# Autodesk Inventor assembly: LowerBody_MIR
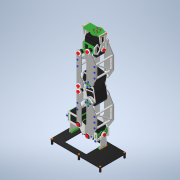
[picture p0: Inventor's stored thumbnail of the model, 180x180]
Saved by Autodesk Inventor 2020 (Build 240168000, 168)
## iProperties
Created: 2021-12-27
Part Number: LowerBody_MIR
Document SubType Name: Assembly
Designer: Masato Kubotera
Mass: 734.319 g
Surface Area: 2704.73 cm^2
Volume: 452.645 cm^3
Density: 1.62229 g/cm^3
Author: Masato Kubotera
## Documents named in this file (12)
- C:\Users\Masato\Desktop\OpenPlatform_ver3_0 - Ver4_1branch\LowerBody\LowerBody_MIR.iam
- C:\Users\Masato\Desktop\OpenPlatform_ver3_0 - Ver4_1branch\LowerBody\Leg_joit\Leg_joint_roll_yaw.iam
- C:\Users\Masato\Desktop\OpenPlatform_ver3_0 - Ver4_1branch\LowerBody\Leg_joit\Leg_joint_roll_pitch.iam
- C:\Users\Masato\Desktop\OpenPlatform_ver3_0 - Ver4_1branch\LowerBody\Slider_crank\Slider_crank_mechanism.iam
- C:\Users\Masato\Desktop\OpenPlatform_ver3_0 - Ver4_1branch\LowerBody\Link\FrontLink.iam
- C:\Users\Masato\Desktop\OpenPlatform_ver3_0 - Ver4_1branch\LowerBody\Link\BackUpperLink.iam
- C:\Users\Masato\Desktop\OpenPlatform_ver3_0 - Ver4_1branch\LowerBody\Link\BackLowerLink.iam
- C:\Users\Masato\Desktop\OpenPlatform_ver3_0 - Ver4_1branch\LowerBody\Ankle\Ankle_side_pitch.iam
- C:\Users\Masato\Desktop\OpenPlatform_ver3_0 - Ver4_1branch\Ready_Made\Screw\M2_6-8.ipt
- C:\Users\Masato\Desktop\OpenPlatform_ver3_0 - Ver4_1branch\LowerBody\Knee\Knee_MIR.iam
- C:\Users\Masato\Desktop\OpenPlatform_ver3_0 - Ver4_1branch\LowerBody\Ankle\Ankle_MIR.iam
- C:\Users\Masato\Desktop\OpenPlatform_ver3_0 - Ver4_1branch\LowerBody\Foot\Foot_MIR.iam
## Components (20 placed, 11 different names)
1. Leg_joint_roll_yaw:1 [sub-assembly] — 角度:1【付け根ロール軸】, 挿入:2, 挿入:1, フラッシュ:2, メイト:1, フラッシュ:1, 角度:2
2. Leg_joint_roll_pitch:1 [sub-assembly] — 角度:1【付け根ロール軸】, 挿入:2, 挿入:1, 挿入:7, 挿入:5, 挿入:3, 挿入:6, 挿入:4
3. Slider_crank_mechanism:1 [sub-assembly] — 挿入:3, 角度:2
4. FrontLink:1 [sub-assembly] — 挿入:6, 角度:3, 挿入:4, 挿入:20, 角度:5【膝上ピッチ】
5. BackUpperLink:1 [sub-assembly] — 挿入:7, 挿入:5, 角度:3, 挿入:21
6. FrontLink:2 [sub-assembly] — 挿入:10, 挿入:8, 角度:5, 挿入:22, 角度:6【膝下ピッチ】
7. BackLowerLink:1 [sub-assembly] — 挿入:11, 挿入:9, 角度:5, 挿入:23
8. Ankle_side_pitch:1 [sub-assembly] — 挿入:9, 挿入:8, 挿入:12, 挿入:13, 挿入:14, 挿入:15, 角度:7【足首ピッチ】
9. Ankle_side_pitch:2 [sub-assembly] — 挿入:11, 挿入:10, 挿入:16, 挿入:17, 挿入:18, 挿入:19, 挿入:24
10. M2_6-8:1 — 挿入:12
11. M2_6-8:2 — 挿入:13
12. M2_6-8:3 — 挿入:14
13. M2_6-8:4 — 挿入:15
14. M2_6-8:5 — 挿入:16
15. M2_6-8:6 — 挿入:17
16. M2_6-8:7 — 挿入:18
17. M2_6-8:8 — 挿入:19
18. Knee_MIR:1 [sub-assembly] — 挿入:20, 挿入:21, 挿入:22, 挿入:23, 角度:5【膝上ピッチ】, 角度:6【膝下ピッチ】
19. Ankle_MIR:1 [sub-assembly] — 挿入:24, 挿入:25, 角度:7【足首ピッチ】, 角度:8【足首ロール】
20. Foot_MIR:1 [sub-assembly] — 挿入:25, 角度:8【足首ロール】
## Relationships (36: Insert 25, Angle 8, Mate 2, Flush 1)
- 角度:1【付け根ロール軸】 [Angle] (0 deg): Leg_joint_roll_yaw:1 ↔ Leg_joint_roll_pitch:1
- 挿入:2 [Insert]: Leg_joint_roll_yaw:1 ↔ Leg_joint_roll_pitch:1
- 挿入:1 [Insert]: Leg_joint_roll_yaw:1 ↔ Leg_joint_roll_pitch:1
- フラッシュ:2 [Flush]: Leg_joint_roll_yaw:1
- メイト:1 [Mate]: Leg_joint_roll_yaw:1
- フラッシュ:1 [Mate]: Leg_joint_roll_yaw:1
- 挿入:11 [Insert]: BackLowerLink:1 ↔ Ankle_side_pitch:2
- 挿入:9 [Insert]: BackLowerLink:1 ↔ Ankle_side_pitch:1
- 挿入:7 [Insert]: Leg_joint_roll_pitch:1 ↔ BackUpperLink:1
- 挿入:5 [Insert]: Leg_joint_roll_pitch:1 ↔ BackUpperLink:1
- 挿入:10 [Insert]: FrontLink:2 ↔ Ankle_side_pitch:2
- 挿入:8 [Insert]: FrontLink:2 ↔ Ankle_side_pitch:1
- 角度:5 [Angle] (0 deg): FrontLink:2 ↔ BackLowerLink:1
- 挿入:3 [Insert]: Leg_joint_roll_pitch:1 ↔ Slider_crank_mechanism:1
- 角度:2 [Angle] (0 deg): Leg_joint_roll_yaw:1 ↔ Slider_crank_mechanism:1
- 挿入:6 [Insert]: Leg_joint_roll_pitch:1 ↔ FrontLink:1
- 角度:3 [Angle] (0 deg): FrontLink:1 ↔ BackUpperLink:1
- 挿入:4 [Insert]: Leg_joint_roll_pitch:1 ↔ FrontLink:1
- 挿入:12 [Insert]: Ankle_side_pitch:1 ↔ M2_6-8:1
- 挿入:13 [Insert]: Ankle_side_pitch:1 ↔ M2_6-8:2
- 挿入:14 [Insert]: Ankle_side_pitch:1 ↔ M2_6-8:3
- 挿入:15 [Insert]: Ankle_side_pitch:1 ↔ M2_6-8:4
- 挿入:16 [Insert]: Ankle_side_pitch:2 ↔ M2_6-8:5
- 挿入:17 [Insert]: Ankle_side_pitch:2 ↔ M2_6-8:6
- 挿入:18 [Insert]: Ankle_side_pitch:2 ↔ M2_6-8:7
- 挿入:19 [Insert]: Ankle_side_pitch:2 ↔ M2_6-8:8
- 挿入:20 [Insert]: FrontLink:1 ↔ Knee_MIR:1
- 挿入:21 [Insert]: BackUpperLink:1 ↔ Knee_MIR:1
- 挿入:22 [Insert]: FrontLink:2 ↔ Knee_MIR:1
- 挿入:23 [Insert]: BackLowerLink:1 ↔ Knee_MIR:1
- 挿入:24 [Insert]: Ankle_side_pitch:2 ↔ Ankle_MIR:1
- 挿入:25 [Insert]: Ankle_MIR:1 ↔ Foot_MIR:1
- 角度:5【膝上ピッチ】 [Angle] (0 deg): FrontLink:1 ↔ Knee_MIR:1
- 角度:6【膝下ピッチ】 [Angle] (0 deg): FrontLink:2 ↔ Knee_MIR:1
- 角度:7【足首ピッチ】 [Angle] (0 deg): Ankle_side_pitch:1 ↔ Ankle_MIR:1
- 角度:8【足首ロール】 [Angle] (0 deg): Ankle_MIR:1 ↔ Foot_MIR:1
